# Autodesk Inventor assembly: HM1_FIXT1
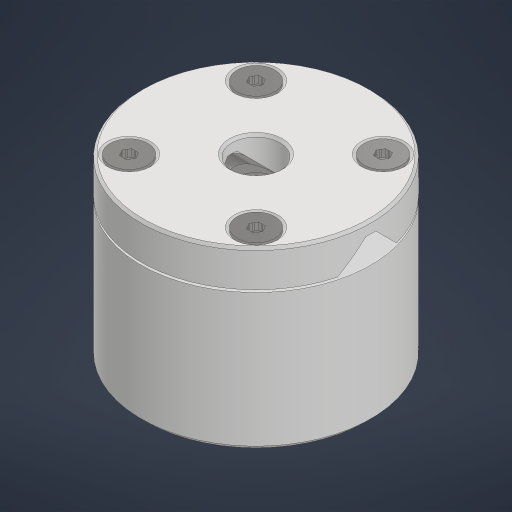
[picture p0: Inventor's stored thumbnail of the model, 512x512]
Saved by Autodesk Inventor 2024.3 (Build 283343000, 343)
## iProperties
Created: 2024-08-19
Part Number: HM1_FIXT1
Document SubType Name: Assembly
Designer: fablabadmin
Author: fablabadmin
## Documents named in this file (5)
- C:\Users\fablabadmin\Documents\_Benjamin_S\_3dCAD\HHVerkstad\Hammer1\_FIXT\HM1_FIXT1.iam
- C:\Users\fablabadmin\Documents\_Benjamin_S\_3dCAD\HHVerkstad\Hammer1\_FIXT\HM1_FIXT1-001.ipt
- C:\Users\fablabadmin\Documents\_Benjamin_S\_3dCAD\HHVerkstad\Hammer1\HM1-002.ipt
- C:\Users\fablabadmin\Documents\_Benjamin_S\_3dCAD\HHVerkstad\Hammer1\_FIXT\HM1_FIXT1-002.ipt
- C:\Users\fablabadmin\Documents\Inventor\Content Center Files\R2024\en-US\ASME ANSI B18.3.5M(2)\ASME_ANSI B18.3.5M - M8x30(2).ipt
## Components (7 placed, 4 different names)
1. HM1_FIXT1-001:1 — Mate:1, Angle:1, Tangent:1, Mate:2
2. HM1_FIXT1-002:1 — Mate:2, Tangent:2, Mate:4, Mate:5, Mate:6, Mate:7
3. HM1-002:1 — Mate:1, Angle:1, Tangent:1, Tangent:2
4. Broached Hexagon Socket Flat Countersunk Head Cap Screws - Metric M8x30:1 — Mate:4
5. Broached Hexagon Socket Flat Countersunk Head Cap Screws - Metric M8x30:2 — Mate:5
6. Broached Hexagon Socket Flat Countersunk Head Cap Screws - Metric M8x30:3 — Mate:6
7. Broached Hexagon Socket Flat Countersunk Head Cap Screws - Metric M8x30:4 — Mate:7
## Relationships (9: Mate 6, Tangent 2, Angle 1)
- Mate:1: HM1_FIXT1-001:1 ↔ HM1-002:1
- Angle:1 (0 deg): HM1_FIXT1-001:1 ↔ HM1-002:1
- Tangent:1: HM1_FIXT1-001:1 ↔ HM1-002:1
- Mate:2: HM1_FIXT1-001:1 ↔ HM1_FIXT1-002:1
- Tangent:2: HM1_FIXT1-002:1 ↔ HM1-002:1
- Mate:4: HM1_FIXT1-002:1 ↔ Broached Hexagon Socket Flat Countersunk Head Cap Screws - Metric M8x30:1
- Mate:5: HM1_FIXT1-002:1 ↔ Broached Hexagon Socket Flat Countersunk Head Cap Screws - Metric M8x30:2
- Mate:6: HM1_FIXT1-002:1 ↔ Broached Hexagon Socket Flat Countersunk Head Cap Screws - Metric M8x30:3
- Mate:7: HM1_FIXT1-002:1 ↔ Broached Hexagon Socket Flat Countersunk Head Cap Screws - Metric M8x30:4
